# Autodesk Inventor assembly: mascon-new
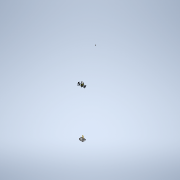
[picture p0: Inventor's stored thumbnail of the model, 180x180]
Saved by Autodesk Inventor 2021 (Build 250183000, 183)
## iProperties
Created: 2021-04-28
Part Number: mascon-new
Document SubType Name: Assembly
Designer: ben
Author: ben
## Documents named in this file (5)
- C:\Users\teh18\OneDrive\BVE Controller\r68-bve-mascon\mascon-new.iam
- C:\Users\teh18\OneDrive\BVE Controller\r68-bve-mascon\handle-base\handle-base.iam
- C:\Users\teh18\OneDrive\BVE Controller\r68-bve-mascon\handle\handle.iam
- C:\Users\teh18\OneDrive\BVE Controller\r68-bve-mascon\shell\shell.iam
- C:\Users\teh18\OneDrive\BVE Controller\r68-bve-mascon\handle_base2.ipt
## Components (4 placed, 4 different names)
1. handle-base:1 [sub-assembly] — handle pop, Flush:1
2. handle:1 [sub-assembly] — handle pop
3. shell:1 [sub-assembly] — Mate:1, Mate:2
4. handle_base2:1 — Flush:1, Mate:1, Mate:2
## Relationships (4: Mate 2, RevoluteJoint 1, Flush 1)
- handle pop [RevoluteJoint]: handle-base:1 ↔ handle:1
- Flush:1: handle-base:1 ↔ handle_base2:1
- Mate:1: shell:1 ↔ handle_base2:1
- Mate:2: shell:1 ↔ handle_base2:1
